# Autodesk Inventor assembly: PortaPiezas
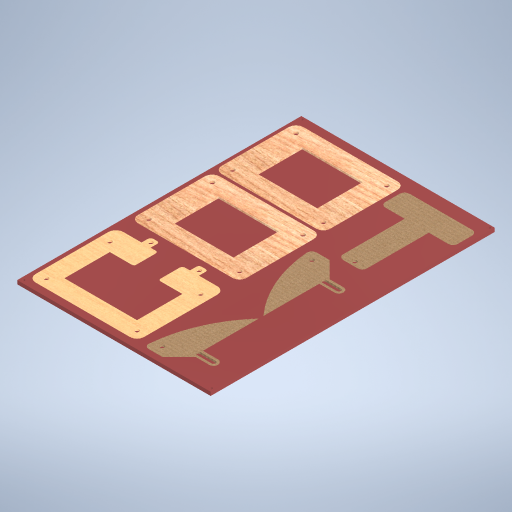
[picture p0: Inventor's stored thumbnail of the model, 512x512]
Saved by Autodesk Inventor 2023.1 (Build 271208000, 208)
## iProperties
Created: 2022-11-11
Part Number: PortaPiezas
Document SubType Name: Assembly
Designer: Daniel Peña
Author: Daniel Peña
## Documents named in this file (7)
- E:\Daniel DiscoA\Documents\UNAL\ProyectoRobotica\CAD\V3 - BigChungus\PortaPiezas.iam
- E:\Daniel DiscoA\Documents\UNAL\ProyectoRobotica\CAD\V3 - BigChungus\Base.ipt
- E:\Daniel DiscoA\Documents\UNAL\ProyectoRobotica\CAD\MarcoRompecabezas.ipt
- E:\Daniel DiscoA\Documents\UNAL\ProyectoRobotica\CAD\V3 - BigChungus\MarcoBC.ipt
- E:\Daniel DiscoA\Documents\UNAL\ProyectoRobotica\CAD\V3 - BigChungus\PistonBC.ipt
- E:\Daniel DiscoA\Documents\UNAL\ProyectoRobotica\CAD\V3 - BigChungus\TapaBC.ipt
- E:\Daniel DiscoA\Documents\UNAL\ProyectoRobotica\CAD\V3 - BigChungus\Dedo-BC.ipt
## Components (8 placed, 6 different names)
1. Base:1 — Flush:1, Insert:1, Insert:2, Insert:3, Insert:4, Mate:13, Mate:14, Mate:15, Mate:16, Mate:17, Mate:18
2. MarcoRompecabezas:1 — Flush:1, Insert:1, Insert:2, Insert:3, Insert:4, Mate:1, Mate:2, Mate:3, Mate:4, Mate:5, Mate:6, Mate:7, Mate:8, Mate:9, Mate:10, Mate:11, Mate:12
3. MarcoBC:1 — Mate:1, Mate:2, Mate:13
4. PistonBC:1 — Mate:11, Mate:12, Mate:16
5. TapaBC:1 — Mate:3, Mate:4, Mate:14
6. TapaBC:2 — Mate:5, Mate:6, Mate:15
7. Dedo-BC:1 — Mate:7, Mate:8, Mate:18
8. Dedo-BC:2 — Mate:9, Mate:10, Mate:17
## Relationships (23: Mate 18, Insert 4, Flush 1)
- Flush:1: Base:1 ↔ MarcoRompecabezas:1
- Insert:1: Base:1 ↔ MarcoRompecabezas:1
- Insert:2: Base:1 ↔ MarcoRompecabezas:1
- Insert:3: Base:1 ↔ MarcoRompecabezas:1
- Insert:4: Base:1 ↔ MarcoRompecabezas:1
- Mate:1: MarcoRompecabezas:1 ↔ MarcoBC:1
- Mate:2: MarcoRompecabezas:1 ↔ MarcoBC:1
- Mate:3: MarcoRompecabezas:1 ↔ TapaBC:1
- Mate:4: MarcoRompecabezas:1 ↔ TapaBC:1
- Mate:5: MarcoRompecabezas:1 ↔ TapaBC:2
- Mate:6: MarcoRompecabezas:1 ↔ TapaBC:2
- Mate:7: MarcoRompecabezas:1 ↔ Dedo-BC:1
- Mate:8: MarcoRompecabezas:1 ↔ Dedo-BC:1
- Mate:9: MarcoRompecabezas:1 ↔ Dedo-BC:2
- Mate:10: MarcoRompecabezas:1 ↔ Dedo-BC:2
- Mate:11: MarcoRompecabezas:1 ↔ PistonBC:1
- Mate:12: MarcoRompecabezas:1 ↔ PistonBC:1
- Mate:13: Base:1 ↔ MarcoBC:1
- Mate:14: Base:1 ↔ TapaBC:1
- Mate:15: Base:1 ↔ TapaBC:2
- Mate:16: Base:1 ↔ PistonBC:1
- Mate:17: Base:1 ↔ Dedo-BC:2
- Mate:18: Base:1 ↔ Dedo-BC:1
